# Autodesk Inventor assembly: DiaD Side Bumper
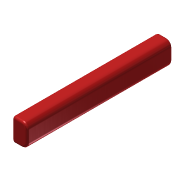
[picture p0: Inventor's stored thumbnail of the model, 180x180]
Saved by Autodesk Inventor 2013 (Build 170138000, 138)
## iProperties
Created: 2013-05-20
Part Number: DiaD Side Bumper
Document SubType Name: Assembly
Designer: Nemo
Author: Nemo
## Documents named in this file (6)
- H:\Nemo\Documents\Robotics\COTS Parts\Drive in a Day\DiaD Side Bumper.iam
- H:\Nemo\Documents\Robotics\COTS Parts\Drive in a Day\217-2593-015 Rev2 Bumper Mount Side.ipt
- H:\Nemo\Documents\Robotics\COTS Parts\Drive in a Day\SideBumpers.ipt
- H:\Nemo\Documents\Robotics\COTS Parts\Drive in a Day\DiaD bumper fastener subassy.iam
- H:\Nemo\Documents\Robotics\COTS Parts\Fasteners\14-20 locknut.ipt
- H:\Nemo\Documents\Robotics\COTS Parts\Fasteners\14-20 BHCS x750.ipt
## Components (15 placed, 5 different names)
1. 217-2593-015 Rev2 Bumper Mount Side:1 — Insert:1, Insert:2, Insert:15, Insert:16, Insert:17, Insert:18
2. 217-2593-015 Rev2 Bumper Mount Side:2 — Insert:3, Insert:4, Insert:19, Insert:20, Insert:21, Insert:22
3. SideBumpers:1
4. DiaD bumper fastener subassy:1 [sub-assembly] — Insert:1
5. DiaD bumper fastener subassy:2 [sub-assembly] — Insert:2
6. DiaD bumper fastener subassy:3 [sub-assembly] — Insert:3
7. DiaD bumper fastener subassy:4 [sub-assembly] — Insert:4
8. 14-20 BHCS x750:4 — Insert:17
9. 14-20 locknut:4 — Insert:16
10. 14-20 BHCS x750:3 — Insert:15
11. 14-20 locknut:5 — Insert:18
12. 14-20 BHCS x750:2 — Insert:20
13. 14-20 locknut:6 — Insert:19
14. 14-20 locknut:7 — Insert:22
15. 14-20 BHCS x750:1 — Insert:21
## Relationships (13: Insert 12, Mate 1)
- [Mate]: 217-2593-015 Rev2 Bumper Mount Side:1 ↔ SideBumpers:1
- Insert:1: 217-2593-015 Rev2 Bumper Mount Side:1 ↔ DiaD bumper fastener subassy:1
- Insert:2: 217-2593-015 Rev2 Bumper Mount Side:1 ↔ DiaD bumper fastener subassy:2
- Insert:3: 217-2593-015 Rev2 Bumper Mount Side:2 ↔ DiaD bumper fastener subassy:3
- Insert:4: 217-2593-015 Rev2 Bumper Mount Side:2 ↔ DiaD bumper fastener subassy:4
- Insert:15: 217-2593-015 Rev2 Bumper Mount Side:1 ↔ 14-20 BHCS x750:3
- Insert:16 (3.175 mm): 217-2593-015 Rev2 Bumper Mount Side:1 ↔ 14-20 locknut:4
- Insert:17: 217-2593-015 Rev2 Bumper Mount Side:1 ↔ 14-20 BHCS x750:4
- Insert:18 (4.445 mm): 217-2593-015 Rev2 Bumper Mount Side:1 ↔ 14-20 locknut:5
- Insert:19 (4.445 mm): 217-2593-015 Rev2 Bumper Mount Side:2 ↔ 14-20 locknut:6
- Insert:20: 217-2593-015 Rev2 Bumper Mount Side:2 ↔ 14-20 BHCS x750:2
- Insert:21: 217-2593-015 Rev2 Bumper Mount Side:2 ↔ 14-20 BHCS x750:1
- Insert:22 (3.175 mm): 217-2593-015 Rev2 Bumper Mount Side:2 ↔ 14-20 locknut:7
